# Autodesk Inventor assembly: Assembly1
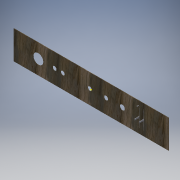
[picture p0: Inventor's stored thumbnail of the model, 180x180]
Saved by Autodesk Inventor 2017 (Build 210142000, 142)
## iProperties
Created: 2017-03-31
Part Number: Assembly1
Document SubType Name: Assembly
Designer: plumbj
Author: plumbj
## Documents named in this file (4)
- C:\Users\plumbj\Desktop\TSI\Rack Plate Inventor\Assembly1.iam
- C:\Users\plumbj\Desktop\TSI\Rack Plate Inventor\Faceplate.ipt
- C:\Users\plumbj\Desktop\TSI\Rack Plate Inventor\pta4543-2x15cpxxxx.ipt
- C:\Users\plumbj\Desktop\TSI\Rack Plate Inventor\92095A452_18-8 SS BUTTON-HEAD SOCKET CAP SCREW.ipt
## Components (4 placed, 3 different names)
1. pta4543-2x15cpxxxx:1 — Mate:1, Flush:1
2. pta4543-2x15cpxxxx:2 — Mate:2, Flush:2
3. Faceplate:1 — Mate:1, Flush:1, Mate:2, Flush:2
4. 92095A452_18-8 SS BUTTON-HEAD SOCKET CAP SCREW:1
## Relationships (4: Mate 2, Flush 2)
- Mate:1: pta4543-2x15cpxxxx:1 ↔ Faceplate:1
- Flush:1: pta4543-2x15cpxxxx:1 ↔ Faceplate:1
- Mate:2: pta4543-2x15cpxxxx:2 ↔ Faceplate:1
- Flush:2: pta4543-2x15cpxxxx:2 ↔ Faceplate:1
